# Autodesk Inventor assembly: Leadscrew Constraint Rear for 4040 - Assembly
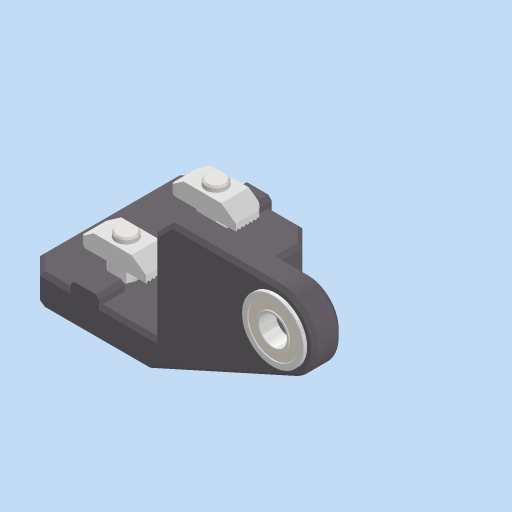
[picture p0: Inventor's stored thumbnail of the model, 512x512]
Saved by Autodesk Inventor 2023.2 (Build 272271000, 271)
## iProperties
Created: 2023-11-23
Part Number: Leadscrew Constraint Rear for 4040 - Assembly
Document SubType Name: Assembly
Designer: Nils Bade
Author: Nils Bade
## Documents named in this file (5)
- C:\Users\nilsb\Documents\Inventor\Projektarbeit-Bade\RatRig_modified\Leadscrew Constraint Rear for 4040 - Assembly.iam
- C:\Users\nilsb\Documents\Inventor\Projektarbeit-Bade\RatRig_modified\Leadscrew Constraint Rear for 4040.ipt
- C:\Users\nilsb\Documents\Inventor\Projektarbeit-Bade\RatRig_modified\T-NUT - DropIn 4040 SERIES - M6.ipt
- C:\Users\nilsb\Documents\Inventor\Projektarbeit-Bade\Schrauben\Cap Head Screw M6x16.ipt
- C:\Users\nilsb\Documents\Inventor\Projektarbeit-Bade\RatRig_Standards\Ball Bearing - F688ZZ v1.ipt
## Components (6 placed, 4 different names)
1. Leadscrew Constraint Rear 4040:1 — Passend:5, Passend:6, Winkel:1, Winkel:2, Passend:13, Passend:14, Passend:15, Passend:16, Passend:19, Passend:20
2. T-NUT - DROP IN TYPE FOR 40 SERIES - M6:1 — Passend:5, Winkel:1, Passend:18
3. T-NUT - DROP IN TYPE FOR 40 SERIES - M6:2 — Passend:6, Winkel:2, Passend:17
4. Cap Head Screw M6x16:1 — Passend:15, Passend:18, Passend:19
5. Cap Head Screw M6x16:2 — Passend:16, Passend:17, Passend:20
6. Ball Bearing - F688ZZ v1:1 — Passend:13, Passend:14
## Relationships (12: Mate 10, Angle 2)
- Passend:5 [Mate] (4.5 mm): Leadscrew Constraint Rear 4040:1 ↔ T-NUT - DROP IN TYPE FOR 40 SERIES - M6:1
- Passend:6 [Mate] (4.5 mm): Leadscrew Constraint Rear 4040:1 ↔ T-NUT - DROP IN TYPE FOR 40 SERIES - M6:2
- Winkel:1 [Angle] (0 deg): Leadscrew Constraint Rear 4040:1 ↔ T-NUT - DROP IN TYPE FOR 40 SERIES - M6:1
- Winkel:2 [Angle] (0 deg): Leadscrew Constraint Rear 4040:1 ↔ T-NUT - DROP IN TYPE FOR 40 SERIES - M6:2
- Passend:13 [Mate]: Leadscrew Constraint Rear 4040:1 ↔ Ball Bearing - F688ZZ v1:1
- Passend:14 [Mate]: Leadscrew Constraint Rear 4040:1 ↔ Ball Bearing - F688ZZ v1:1
- Passend:15 [Mate]: Leadscrew Constraint Rear 4040:1 ↔ Cap Head Screw M6x16:1
- Passend:16 [Mate]: Leadscrew Constraint Rear 4040:1 ↔ Cap Head Screw M6x16:2
- Passend:17 [Mate]: T-NUT - DROP IN TYPE FOR 40 SERIES - M6:2 ↔ Cap Head Screw M6x16:2
- Passend:18 [Mate]: T-NUT - DROP IN TYPE FOR 40 SERIES - M6:1 ↔ Cap Head Screw M6x16:1
- Passend:19 [Mate]: Leadscrew Constraint Rear 4040:1 ↔ Cap Head Screw M6x16:1
- Passend:20 [Mate]: Leadscrew Constraint Rear 4040:1 ↔ Cap Head Screw M6x16:2
